# Autodesk Inventor assembly: gaming controllbox
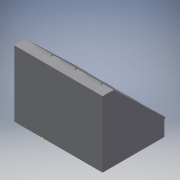
[picture p0: Inventor's stored thumbnail of the model, 180x180]
Saved by Autodesk Inventor 2016 (Build 200138000, 138)
## iProperties
Created: 2016-05-17
Part Number: gaming controllbox
Document SubType Name: Assembly
Designer: Lillahunden
Author: Lillahunden
## Documents named in this file (7)
- C:\Users\Lillahunden\Documents\Inventor\Gaming controllbox\gaming controllbox.iam
- C:\Users\Lillahunden\Documents\Inventor\Gaming controllbox\bottom.ipt
- C:\Users\Lillahunden\Documents\Inventor\Gaming controllbox\back.ipt
- C:\Users\Lillahunden\Documents\Inventor\Gaming controllbox\top.ipt
- C:\Users\Lillahunden\Documents\Inventor\Gaming controllbox\front.ipt
- C:\Users\Lillahunden\Documents\Inventor\Gaming controllbox\left.ipt
- C:\Users\Lillahunden\Documents\Inventor\Gaming controllbox\Frontpanel.ipt
## Components (7 placed, 6 different names)
1. bottom:1 — Mate:1, Flush:1, Flush:3, Flush:4, Flush:6
2. back:1 — Mate:1, Flush:1, Flush:2, Flush:7
3. top:1 — Flush:2
4. front:1 — Flush:3, Flush:5
5. left:1 — Flush:4, Flush:8
6. left:2 — Flush:5, Flush:6, Flush:7
7. Frontpanel:1 — Flush:8
## Relationships (9: Flush 8, Mate 1)
- Mate:1: bottom:1 ↔ back:1
- Flush:1: bottom:1 ↔ back:1
- Flush:2: back:1 ↔ top:1
- Flush:3: bottom:1 ↔ front:1
- Flush:4: bottom:1 ↔ left:1
- Flush:5: front:1 ↔ left:2
- Flush:6: bottom:1 ↔ left:2
- Flush:7: back:1 ↔ left:2
- Flush:8: left:1 ↔ Frontpanel:1
